# Autodesk Inventor assembly: 276-2174
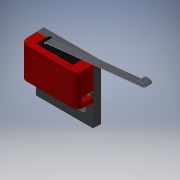
[picture p0: Inventor's stored thumbnail of the model, 180x180]
Saved by Autodesk Inventor 2019.4 (Build 234330000, 330)
## iProperties
Category: Sensors
Company: Autodesk Inc.
Created: 2012-04-10
Part Number: 276-2174
Document SubType Name: Assembly
Catalog Web Link: http://www.vexrobotics.com/products/accessories/sensors/276-2174.html
Vendor: VEX
Designer: Autodesk Inc.
Mass: 6.09491 g
Surface Area: 67.6161 cm^2
Volume: 5.82641 cm^3
Density: 1.04608 g/cm^3
Author: Autodesk Inc.
## Documents named in this file (4)
- D:\towerTakeOverCad\cadlib\传感器\Limit Switch.iam
- D:\towerTakeOverCad\cadlib\传感器\Reference Parts\Limit Switch\Microswitch.ipt
- D:\towerTakeOverCad\cadlib\传感器\Reference Parts\Limit Switch\Bottom.ipt
- D:\towerTakeOverCad\cadlib\传感器\Reference Parts\Limit Switch\Top.ipt
## Components (3 placed, 3 different names)
1. Microswitch:1 — Mate:5, Mate:6, Mate:7
2. Bottom:1 — Mate:1, Mate:2, Insert:1, Insert:2, Mate:5, Mate:6, Mate:7
3. Top:1 — Insert:1, Insert:2
## Relationships (9: Mate 7, Insert 2)
- Mate:1: Bottom:1
- Mate:2: Bottom:1
- Mate:3
- Mate:4
- Insert:1: Bottom:1 ↔ Top:1
- Insert:2: Bottom:1 ↔ Top:1
- Mate:5: Microswitch:1 ↔ Bottom:1
- Mate:6: Microswitch:1 ↔ Bottom:1
- Mate:7: Microswitch:1 ↔ Bottom:1
